# Autodesk Inventor assembly: bras_main
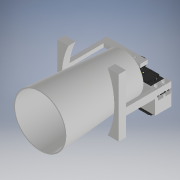
[picture p0: Inventor's stored thumbnail of the model, 180x180]
Saved by Autodesk Inventor 2020 (Build 240168000, 168)
## iProperties
Created: 2019-12-27
Part Number: bras_main
Document SubType Name: Assembly
Designer: bapti
Author: bapti
## Documents named in this file (5)
- C:\Users\bapti\Documents\EIRBOT\eirbot2020-2A\Meca\EIRBOT_sailtheworld\robot\bras\bras_main.iam
- C:\Users\bapti\Documents\EIRBOT\eirbot2020-2A\Meca\EIRBOT_sailtheworld\mg995\MG_996R.iam
- C:\Users\bapti\Documents\EIRBOT\eirbot2020-2A\Meca\EIRBOT_sailtheworld\board\boue.ipt
- C:\Users\bapti\Documents\EIRBOT\eirbot2020-2A\Meca\EIRBOT_sailtheworld\robot\bras\pince_mouvante.ipt
- C:\Users\bapti\Documents\EIRBOT\eirbot2020-2A\Meca\EIRBOT_sailtheworld\robot\bras\pince_statique.ipt
## Components (4 placed, 4 different names)
1. MG_996R:1 [sub-assembly] — Affleurement:1, Affleurement:2, Affleurement:3, Placage:1, Placage:2, Placage:3, Placage:4, Placage:5
2. boue:1
3. pince_mouvante:1 — Placage:4, Placage:5
4. pince_statique:1 — Placage:1, Placage:2, Placage:3
## Relationships (8: Mate 5, Flush 3)
- Affleurement:1 [Flush]: MG_996R:1
- Affleurement:2 [Flush]: MG_996R:1
- Affleurement:3 [Flush]: MG_996R:1
- Placage:1 [Mate]: MG_996R:1 ↔ pince_statique:1
- Placage:2 [Mate]: MG_996R:1 ↔ pince_statique:1
- Placage:3 [Mate]: MG_996R:1 ↔ pince_statique:1
- Placage:4 [Mate]: MG_996R:1 ↔ pince_mouvante:1
- Placage:5 [Mate]: MG_996R:1 ↔ pince_mouvante:1
